# Autodesk Inventor assembly: TR1 Actuator
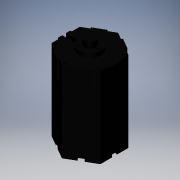
[picture p0: Inventor's stored thumbnail of the model, 180x180]
Saved by Autodesk Inventor 2017 (Build 210142000, 142)
## iProperties
Created: 2018-10-09
Part Number: TR1 Actuator
Document SubType Name: Assembly
Designer: Zach
Author: Zach
## Documents named in this file (17)
- C:\Users\Dell\Documents\GitHub\tr2\Arm Actuator\Arm Actuator.iam
- C:\Users\Dell\Documents\GitHub\tr2\Arm Actuator\TA01.ipt
- C:\Users\Dell\Documents\GitHub\tr2\Arm Actuator\Arm Actuator\Design Accelerator\Spur Gears2.iam
- C:\Users\Dell\Documents\GitHub\tr2\Arm Actuator\Arm Actuator\Design Accelerator\Spur Gears3.iam
- C:\Users\Dell\Documents\GitHub\tr2\Arm Actuator\EMS22XXX-D28-LSX.ipt
- C:\Users\Dell\Documents\GitHub\tr2\Arm Actuator\12RPM Gear Motor.ipt
- C:\Users\Dell\Documents\GitHub\tr2\Arm Actuator\Slip Ring.ipt
- C:\Users\Dell\Documents\GitHub\tr2\Arm Actuator\TA06.ipt
- C:\Users\Dell\Documents\GitHub\tr2\Arm Actuator\6mm Mounting Hub, thin.ipt
- C:\Users\Dell\Documents\GitHub\tr2\Arm Actuator\Steel Tubing.ipt
- C:\Users\Dell\Documents\GitHub\tr2\Arm Actuator\Flange Bearing.ipt
- C:\Users\Dell\Documents\GitHub\tr2\Arm Actuator\Shaft Collar.ipt
- C:\Users\Dell\Documents\GitHub\tr2\Arm Actuator\Arm Actuator\Design Accelerator\Spur Gear13.ipt
- C:\Users\Dell\Documents\GitHub\tr2\Arm Actuator\6mm Mounting Hub, thick.ipt
- C:\Users\Dell\Documents\GitHub\tr2\Arm Actuator\TA02c.ipt
- C:\Users\Dell\Documents\GitHub\tr2\Arm Actuator\TA02b.ipt
- C:\Users\Dell\Documents\GitHub\tr2\Arm Actuator\Bushing.ipt
## Components (20 placed, 15 different names)
1. TA01:1 — Mate:108, Mate:109, Mate:110, Mate:111
2. TA06:1 — Mate:34, Mate:35, Mate:36, Mate:82, Mate:83
3. Spur Gears:1 [sub-assembly] — Mate:33, Mate:36, Mate:80, Mate:81, Rotation:1, Rotation:2, Mate:94, Mate:95, Mate:97
4. Spur Gears:4 [sub-assembly] — Mate:23, Mate:54, Rotation:2, Mate:92
5. 12RPM Gear Motor:1 — Mate:86, Mate:88, Mate:102, Mate:103
6. EMS22XXX-D28-LSX:1 — Mate:23, Mate:45, Mate:101
7. Slip Ring:1 — Mate:33, Mate:34, Mate:35, Mate:83
8. 6mm Mounting Hub, thin:1 — Mate:45, Mate:54, Mate:92
9. Steel Tubing:1 — Mate:76, Mate:77, Flush:2, Mate:79, Mate:82, Mate:84, Mate:96, Mate:98, Mate:104
10. Flange Bearing:1 — Mate:76, Mate:78
11. Shaft Collar:1 — Mate:77, Mate:78, Flush:2
12. Shaft Collar:2 — Mate:79, Mate:80, Mate:81
13. Flange Bearing:2 — Mate:84
14. Spur Gear1:1 — Mate:88, Mate:89, Rotation:1
15. 6mm Mounting Hub, thick:1 — Mate:86, Mate:89
16. Flange Bearing:3 — Mate:94, Mate:95
17. TA02c:1 — Mate:98, Mate:99, Mate:100, Mate:105, Mate:108, Mate:109, Mate:110, Mate:111
18. TA02b:1 — Mate:96, Mate:97, Mate:99, Mate:100, Mate:101, Mate:102, Mate:103, Mate:106, Mate:107
19. Bushing:1 — Mate:104, Mate:105
20. Bushing:2 — Mate:106, Mate:107
## Relationships (41: Mate 38, RelateRotation 2, Flush 1)
- Mate:23: Spur Gears:4 ↔ EMS22XXX-D28-LSX:1
- Mate:33: Spur Gears:1 ↔ Slip Ring:1
- Mate:34: TA06:1 ↔ Slip Ring:1
- Mate:35: TA06:1 ↔ Slip Ring:1
- Mate:36: TA06:1 ↔ Spur Gears:1
- Mate:45: EMS22XXX-D28-LSX:1 ↔ 6mm Mounting Hub, thin:1
- Mate:54: Spur Gears:4 ↔ 6mm Mounting Hub, thin:1
- Mate:76: Steel Tubing:1 ↔ Flange Bearing:1
- Mate:77: Steel Tubing:1 ↔ Shaft Collar:1
- Mate:78: Flange Bearing:1 ↔ Shaft Collar:1
- Flush:2: Steel Tubing:1 ↔ Shaft Collar:1
- Mate:79: Steel Tubing:1 ↔ Shaft Collar:2
- Mate:80: Spur Gears:1 ↔ Shaft Collar:2
- Mate:81: Spur Gears:1 ↔ Shaft Collar:2
- Mate:82: TA06:1 ↔ Steel Tubing:1
- Mate:83: TA06:1 ↔ Slip Ring:1
- Mate:84: Steel Tubing:1 ↔ Flange Bearing:2
- Mate:86: 12RPM Gear Motor:1 ↔ 6mm Mounting Hub, thick:1
- Mate:88: 12RPM Gear Motor:1 ↔ Spur Gear1:1
- Mate:89: Spur Gear1:1 ↔ 6mm Mounting Hub, thick:1
- Rotation:1 [RelateRotation] (1 ul): Spur Gears:1 ↔ Spur Gear1:1
- Rotation:2 [RelateRotation] (1 ul): Spur Gears:1 ↔ Spur Gears:4
- Mate:92: Spur Gears:4 ↔ 6mm Mounting Hub, thin:1
- Mate:94: Spur Gears:1 ↔ Flange Bearing:3
- Mate:95: Spur Gears:1 ↔ Flange Bearing:3
- Mate:96: Steel Tubing:1 ↔ TA02b:1
- Mate:97: Spur Gears:1 ↔ TA02b:1
- Mate:98: Steel Tubing:1 ↔ TA02c:1
- Mate:99: TA02c:1 ↔ TA02b:1
- Mate:100: TA02c:1 ↔ TA02b:1
- Mate:101: EMS22XXX-D28-LSX:1 ↔ TA02b:1
- Mate:102: 12RPM Gear Motor:1 ↔ TA02b:1
- Mate:103: 12RPM Gear Motor:1 ↔ TA02b:1
- Mate:104: Steel Tubing:1 ↔ Bushing:1
- Mate:105: TA02c:1 ↔ Bushing:1
- Mate:106: TA02b:1 ↔ Bushing:2
- Mate:107: TA02b:1 ↔ Bushing:2
- Mate:108: TA01:1 ↔ TA02c:1
- Mate:109: TA01:1 ↔ TA02c:1
- Mate:110: TA01:1 ↔ TA02c:1
- Mate:111: TA01:1 ↔ TA02c:1
